# Autodesk Inventor assembly: фуллл
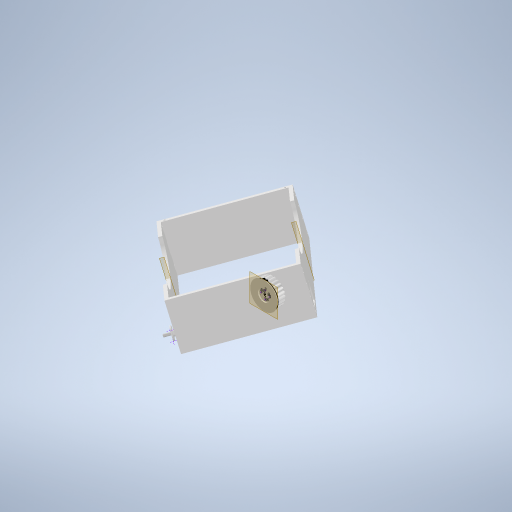
[picture p0: Inventor's stored thumbnail of the model, 512x512]
Saved by Autodesk Inventor 2024.2 (Build 282272000, 272)
## iProperties
Created: 2025-11-20
Part Number: фуллл
Document SubType Name: Assembly
Designer: Zakhar
Author: Zakhar
## Documents named in this file (6)
- C:\Users\Zakhar\Documents\Деталь ВсОШ\Робот.iam
- C:\Users\Zakhar\Documents\Деталь ВсОШ\NEMA17 42-40.ipt
- C:\Users\Zakhar\Documents\Деталь ВсОШ\боковая стенка.ipt
- C:\Users\Zakhar\Documents\Деталь ВсОШ\Муфта.ipt
- C:\Users\Zakhar\Documents\Деталь ВсОШ\передняя стенка.ipt
- C:\Users\Zakhar\Documents\Деталь ВсОШ\Шест.ipt
## Components (7 placed, 5 different names)
1. NEMA17 42-40:1 — Цилиндрический:1, Цилиндрический:2
2. боковая стенка:1 — Жесткий:2, Жесткий:3
3. Муфта:1 — Цилиндрический:2
4. передняя стенка:1 — Жесткий:3
5. Шест:1
6. боковая стенка:2 — Жесткий:1, Цилиндрический:1
7. передняя стенка:2 — Жесткий:1, Жесткий:2
## Relationships (5: WeldJoint 3, CylindricalJoint 2)
- Жесткий:1 [WeldJoint]: боковая стенка:2 ↔ передняя стенка:2
- Жесткий:2 [WeldJoint]: боковая стенка:1 ↔ передняя стенка:2
- Жесткий:3 [WeldJoint]: боковая стенка:1 ↔ передняя стенка:1
- Цилиндрический:1 [CylindricalJoint]: NEMA17 42-40:1 ↔ боковая стенка:2
- Цилиндрический:2 [CylindricalJoint]: NEMA17 42-40:1 ↔ Муфта:1
